# Autodesk Inventor assembly: Ens. Manija
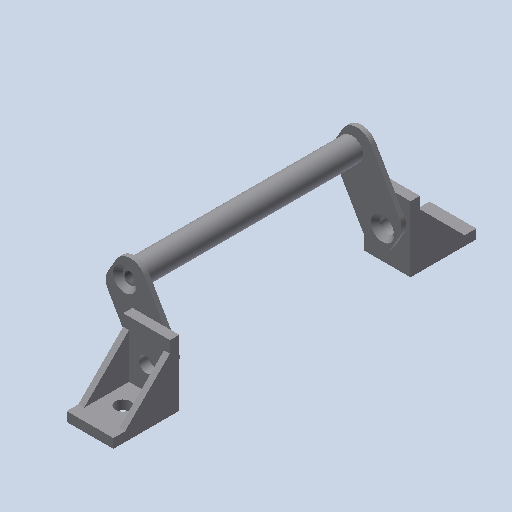
[picture p0: Inventor's stored thumbnail of the model, 512x512]
Saved by Autodesk Inventor 2024.2 (Build 282272000, 272)
## iProperties
Created: 2024-11-25
Part Number: Ens. Manija
Material: Genérico
Document SubType Name: Assembly
Designer: jd.castellanosq
Author: jd.castellanosq
## Documents named in this file (5)
- I:\MICROMECANICA\ALTAS ENERGIAS\Deteccion de Muones\Detectores centelladores\Partes Detector Centellador\SE Matriz Centelladora DC\SSE Manija\SSE. Manija.iam
- I:\MICROMECANICA\ALTAS ENERGIAS\Deteccion de Muones\Detectores centelladores\Partes Detectores centelladores\SSE Manija\Lamina.ipt
- I:\MICROMECANICA\ALTAS ENERGIAS\Deteccion de Muones\Detectores centelladores\Partes Detector Centellador\SE Matriz Centelladora DC\SSE Manija\eje.ipt
- I:\MICROMECANICA\ALTAS ENERGIAS\Deteccion de Muones\Detectores centelladores\Partes Detector Centellador\SE Matriz Centelladora DC\SSE Manija\Escuadra DC.ipt
- I:\MICROMECANICA\ALTAS ENERGIAS\Deteccion de Muones\Detectores centelladores\Partes Detector Centellador\SE Matriz Centelladora DC\SSE Manija\Lamina\Lamina Manija.ipt
## Components (5 placed, 3 different names)
1. eje:1 — Nivelación:1, Nivelación:2, Nivelación:3, Coincidencia:1, Coincidencia:2, Coincidencia:3, Coincidencia:7, Coincidencia:9
2. Escuadra DC:1 — Nivelación:4, Coincidencia:5, Coincidencia:8
3. Escuadra DC:2 — Nivelación:4, Coincidencia:4, Coincidencia:6
4. Lamina Manija:1 — Coincidencia:2, Coincidencia:5, Coincidencia:8, Coincidencia:9
5. Lamina Manija:2 — Coincidencia:3, Coincidencia:4, Coincidencia:6, Coincidencia:7
## Relationships (13: Mate 9, Flush 4)
- Nivelación:1 [Flush]: eje:1
- Nivelación:2 [Flush]: eje:1
- Nivelación:3 [Flush]: eje:1
- Coincidencia:1 [Mate]: eje:1
- Nivelación:4 [Flush]: Escuadra DC:1 ↔ Escuadra DC:2
- Coincidencia:2 [Mate]: eje:1 ↔ Lamina Manija:1
- Coincidencia:3 [Mate]: eje:1 ↔ Lamina Manija:2
- Coincidencia:4 [Mate]: Escuadra DC:2 ↔ Lamina Manija:2
- Coincidencia:5 [Mate]: Escuadra DC:1 ↔ Lamina Manija:1
- Coincidencia:6 [Mate]: Escuadra DC:2 ↔ Lamina Manija:2
- Coincidencia:7 [Mate]: eje:1 ↔ Lamina Manija:2
- Coincidencia:8 [Mate]: Escuadra DC:1 ↔ Lamina Manija:1
- Coincidencia:9 [Mate]: eje:1 ↔ Lamina Manija:1
